# Autodesk Inventor assembly: BrushlessMotor_C5055
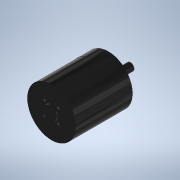
[picture p0: Inventor's stored thumbnail of the model, 180x180]
Saved by Autodesk Inventor 2022.3 (Build 263350000, 350)
## iProperties
Created: 2019-08-30
Part Number: BrushlessMotor_C5055
Document SubType Name: Assembly
Designer: Ryohei
Mass: 454.137 g
Surface Area: 187.891 cm^2
Volume: 115.966 cm^3
Density: 3.91613 g/cm^3
Author: Ryohei
## Documents named in this file (3)
- C:\Users\YusukeKunita\Documents\GrabCAD\Development\BasicParts\BrushlessMotor\BrushlessMotor_C5055.iam
- C:\Users\YusukeKunita\Documents\GrabCAD\Development\BasicParts\BrushlessMotor\Rotar.ipt
- C:\Users\YusukeKunita\Documents\GrabCAD\Development\BasicParts\BrushlessMotor\Stator.ipt
## Components (2 placed, 2 different names)
1. Rotar:1 — 回転:1
2. Stator:1 — 回転:1
## Relationships (1: RevoluteJoint 1)
- 回転:1 [RevoluteJoint]: Rotar:1 ↔ Stator:1
